# Autodesk Inventor assembly: 組合4-17
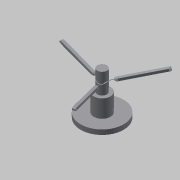
[picture p0: Inventor's stored thumbnail of the model, 180x180]
Saved by Autodesk Inventor 2018 (Build 220112000, 112)
## iProperties
Created: 2021-04-17
Part Number: 組合4-17
Material: 一般
Document SubType Name: Assembly
Designer: 王鼎鈞
Author: 王鼎鈞
## Documents named in this file (5)
- D:\2021顏家民\四人圖檔\組合4-17.iam
- D:\2021顏家民\四人圖檔\支架4-17.ipt
- D:\2021顏家民\四人圖檔\支架4-17-2.ipt
- D:\2021顏家民\四人圖檔\主體4-17.ipt
- D:\2021顏家民\四人圖檔\3d凸輪4-16.ipt
## Components (8 placed, 4 different names)
1. 支架4-17:1 — 貼合:1, 貼合:2, 貼合:3, 相切:1, 相切:2
2. 支架4-17-2:1 — 貼合:1, 貼合:2, 貼合:3, 插入:2
3. 主體4-17:1 — 插入:1, 插入:2, 旋轉:1, 插入:3, 插入:4
4. 3d凸輪4-16:1 — 插入:1, 相切:1, 相切:2, 旋轉:1, 相切:3, 相切:4, 相切:5, 相切:6
5. 支架4-17:2 — 相切:3, 相切:4
6. 支架4-17-2:2 — 插入:4
7. 支架4-17:3 — 相切:5, 相切:6
8. 支架4-17-2:3 — 插入:3
## Relationships (20: Mate 9, Tangent 6, Insert 4, RevoluteJoint 1)
- 貼合:1 [Mate]: 支架4-17:1 ↔ 支架4-17-2:1
- 貼合:2 [Mate]: 支架4-17:1 ↔ 支架4-17-2:1
- 貼合:3 [Mate]: 支架4-17:1 ↔ 支架4-17-2:1
- 插入:1 [Insert]: 主體4-17:1 ↔ 3d凸輪4-16:1
- 插入:2 [Insert]: 支架4-17-2:1 ↔ 主體4-17:1
- 相切:1 [Tangent]: 支架4-17:1 ↔ 3d凸輪4-16:1
- 相切:2 [Tangent]: 支架4-17:1 ↔ 3d凸輪4-16:1
- 旋轉:1 [RevoluteJoint]: 主體4-17:1 ↔ 3d凸輪4-16:1
- [Mate]: 支架4-17:2 ↔ 支架4-17-2:2
- [Mate]: 支架4-17:2 ↔ 支架4-17-2:2
- [Mate]: 支架4-17:2 ↔ 支架4-17-2:2
- [Mate]: 支架4-17:3 ↔ 支架4-17-2:3
- [Mate]: 支架4-17:3 ↔ 支架4-17-2:3
- [Mate]: 支架4-17:3 ↔ 支架4-17-2:3
- 插入:3 [Insert]: 主體4-17:1 ↔ 支架4-17-2:3
- 插入:4 [Insert]: 主體4-17:1 ↔ 支架4-17-2:2
- 相切:3 [Tangent]: 3d凸輪4-16:1 ↔ 支架4-17:2
- 相切:4 [Tangent]: 3d凸輪4-16:1 ↔ 支架4-17:2
- 相切:5 [Tangent]: 3d凸輪4-16:1 ↔ 支架4-17:3
- 相切:6 [Tangent]: 3d凸輪4-16:1 ↔ 支架4-17:3
## Named parameters: d15_d0 = 0 mm, d16_d1 = 0 mm, d17_d2 = 0 mm, d18_d0 = 0 mm, d19_d1 = 0 mm, d20_d2 = 0 mm
